# Autodesk Inventor assembly: fish-drive-proto
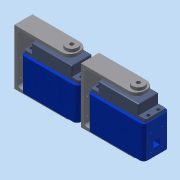
[picture p0: Inventor's stored thumbnail of the model, 180x180]
Saved by Autodesk Inventor 2015 SP1 (Build 190203100, 203)
## iProperties
Created: 2023-12-22
Part Number: fish-drive-proto
Document SubType Name: Assembly
Designer: boss
Author: boss
## Documents named in this file (5)
- Z:\VM-Exchange\work\invp15\UAV\Fish-proto\v01\fish-drive-proto.iam
- Z:\VM-Exchange\work\invp15\UAV\Fish-proto\std\ServoBody.ipt
- Z:\VM-Exchange\work\invp15\UAV\Fish-proto\std\ServoWorkRod.ipt
- Z:\VM-Exchange\work\invp15\UAV\Fish-proto\std\Obolochka.ipt
- Z:\VM-Exchange\work\invp15\UAV\Fish-proto\std\outer-axis.ipt
## Components (8 placed, 4 different names)
1. ServoBody:1
2. ServoWorkRod:1
3. Obolochka:1
4. outer-axis:1
5. ServoBody:2
6. ServoWorkRod:2
7. Obolochka:2
8. outer-axis:2
## Component patterns: (2 elements, first: ServoBody:1 + ServoWorkRod:1 + Obolochka:1 + outer-axis:1)
